# Autodesk Inventor assembly: Handyhalterung
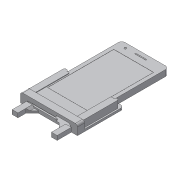
[picture p0: Inventor's stored thumbnail of the model, 180x180]
Saved by Autodesk Inventor 2013 (Build 170138000, 138)
## iProperties
Created: 2013-06-29
Part Number: Handyhalterung
Document SubType Name: Assembly
Designer: Harald
Author: Harald
## Documents named in this file (3)
- C:\Users\Harald\Documents\Inventor\Handyhalterung\Handyhalterung.iam
- C:\Users\Harald\Documents\Inventor\Handyhalterung\Grundplatte.ipt
- C:\Users\Harald\Documents\Inventor\Handyhalterung\Galaxy S2.ipt
## Components (2 placed, 2 different names)
1. Grundplatte:1 — Passend:3, Passend:4, Passend:5
2. Galaxy S2:1 — Passend:3, Passend:4, Passend:5
## Relationships (3: Mate 3)
- Passend:3 [Mate]: Grundplatte:1 ↔ Galaxy S2:1
- Passend:4 [Mate]: Grundplatte:1 ↔ Galaxy S2:1
- Passend:5 [Mate]: Grundplatte:1 ↔ Galaxy S2:1
